# Autodesk Inventor assembly: MO-237
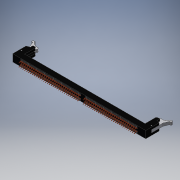
[picture p0: Inventor's stored thumbnail of the model, 180x180]
Saved by Autodesk Inventor 2016 (Build 200138000, 138)
## iProperties
Created: 2016-07-08
Part Number: MO-237
Document SubType Name: Assembly
Designer: Jonathan
Author: Jonathan
## Documents named in this file (4)
- C:\Users\Jonathan\Documents\Projects\mppcInterface\mppcInterface\cad\electronics\MO-237\MO-237.iam
- C:\Users\Jonathan\Documents\Projects\mppcInterface\mppcInterface\cad\electronics\MO-237\body.ipt
- C:\Users\Jonathan\Documents\Projects\mppcInterface\mppcInterface\cad\electronics\MO-237\pins.ipt
- C:\Users\Jonathan\Documents\Projects\mppcInterface\mppcInterface\cad\electronics\MO-237\pins2.ipt
## Components (241 placed, 3 different names)
1. body:1 — Mate:1, Mate:2, Mate:3, Mate:4, Mate:5, Mate:6, Mate:7, Mate:8, Mate:9, Mate:10, Mate:11, Mate:12, Mate:13, Mate:14, Mate:15, Mate:16
2. pins:1 — Mate:1, Mate:2
3. pins:2
4. pins:3
5. pins:4
6. pins:5
7. pins:6
8. pins:7
9. pins:8
10. pins:9
11. pins:10
12. pins:11
13. pins:12
14. pins:13
15. pins:14
16. pins:15
17. pins:16
18. pins:17
19. pins:18
20. pins:19
21. pins:20
22. pins:21
23. pins:22
24. pins:23
25. pins:24
26. pins:25
27. pins:26
28. pins:27
29. pins:28
30. pins:29
31. pins:30
32. pins:31
33. pins:32
34. pins:33 — Mate:3, Mate:4
35. pins:34
36. pins:35
37. pins:36
38. pins:37
39. pins:38
40. pins:39
41. pins:40
42. pins:41
43. pins:42
44. pins:43
45. pins:44
46. pins:45
47. pins:46
48. pins:47
49. pins:48
50. pins:49
51. pins:50
52. pins:51
53. pins:52
54. pins:53
55. pins:54
56. pins:55
57. pins:56
58. pins:57
59. pins:58
60. pins:59
61. pins:60
62. pins:61 — Mate:5, Mate:6
63. pins:62
64. pins:63
65. pins:64
66. pins:65
67. pins:66
68. pins:67
69. pins:68
70. pins:69
71. pins:70
72. pins:71
73. pins:72
74. pins:73
75. pins:74
76. pins:75
77. pins:76
78. pins:77
79. pins:78
80. pins:79
81. pins:80
82. pins:81
83. pins:82
84. pins:83
85. pins:84
86. pins:85
87. pins:86
88. pins:87
89. pins:88
90. pins:89
91. pins:90
92. pins:91
93. pins:92
94. pins:93 — Mate:7, Mate:8
95. pins:94
96. pins:95
97. pins:96
98. pins:97
99. pins:98
100. pins:99
101. pins:100
102. pins:101
103. pins:102
104. pins:103
105. pins:104
106. pins:105
107. pins:106
108. pins:107
109. pins:108
110. pins:109
111. pins:110
112. pins:111
113. pins:112
114. pins:113
115. pins:114
116. pins:115
117. pins:116
118. pins:117
119. pins:118
120. pins:119
121. pins:120
122. pins2:1 — Mate:9, Mate:10
123. pins2:5
124. pins2:6
125. pins2:7
126. pins2:8
127. pins2:9
128. pins2:10
129. pins2:11
130. pins2:12
131. pins2:13
132. pins2:14
133. pins2:15
134. pins2:16
135. pins2:17
136. pins2:18
137. pins2:19
138. pins2:20
139. pins2:21
140. pins2:22
141. pins2:23
142. pins2:24
143. pins2:25
144. pins2:26
145. pins2:27
146. pins2:28
147. pins2:29
148. pins2:30
149. pins2:31
150. pins2:2 — Mate:11, Mate:12
151. pins2:32
152. pins2:33
153. pins2:34
154. pins2:35
155. pins2:36
156. pins2:37
157. pins2:38
158. pins2:39
159. pins2:40
160. pins2:41
161. pins2:42
162. pins2:43
163. pins2:44
164. pins2:45
165. pins2:46
166. pins2:47
167. pins2:48
168. pins2:49
169. pins2:50
170. pins2:51
171. pins2:52
172. pins2:53
173. pins2:54
174. pins2:55
175. pins2:56
176. pins2:57
177. pins2:58
178. pins2:4 — Mate:13, Mate:14
179. pins2:59
180. pins2:60
181. pins2:61
182. pins2:62
183. pins2:63
184. pins2:64
185. pins2:65
186. pins2:66
187. pins2:67
188. pins2:68
189. pins2:69
190. pins2:70
191. pins2:71
192. pins2:72
193. pins2:73
194. pins2:74
195. pins2:75
196. pins2:76
197. pins2:77
198. pins2:78
199. pins2:79
200. pins2:80
201. pins2:81
202. pins2:82
203. pins2:83
204. pins2:84
205. pins2:85
206. pins2:86
207. pins2:87
208. pins2:88
209. pins2:89
210. pins2:3 — Mate:15, Mate:16
211. pins2:90
212. pins2:91
213. pins2:92
214. pins2:93
215. pins2:94
216. pins2:95
217. pins2:96
218. pins2:97
219. pins2:98
220. pins2:99
221. pins2:100
222. pins2:101
223. pins2:102
224. pins2:103
225. pins2:104
226. pins2:105
227. pins2:106
228. pins2:107
229. pins2:108
230. pins2:109
231. pins2:110
232. pins2:111
233. pins2:112
234. pins2:113
235. pins2:114
236. pins2:115
237. pins2:116
238. pins2:117
239. pins2:118
240. pins2:119
241. pins2:120
## Component patterns: (32 elements, first: pins:1), (28 elements, first: pins:33), (32 elements, first: pins:61), (28 elements, first: pins:93), (28 elements, first: pins2:1), (28 elements, first: pins2:2), (32 elements, first: pins2:4), (32 elements, first: pins2:3)
## Relationships (16: Mate 16)
- Mate:1: body:1 ↔ pins:1
- Mate:2: body:1 ↔ pins:1
- Mate:3: body:1 ↔ pins:33
- Mate:4: body:1 ↔ pins:33
- Mate:5: body:1 ↔ pins:61
- Mate:6: body:1 ↔ pins:61
- Mate:7: body:1 ↔ pins:93
- Mate:8: body:1 ↔ pins:93
- Mate:9: body:1 ↔ pins2:1
- Mate:10: body:1 ↔ pins2:1
- Mate:11: body:1 ↔ pins2:2
- Mate:12: body:1 ↔ pins2:2
- Mate:13: body:1 ↔ pins2:4
- Mate:14: body:1 ↔ pins2:4
- Mate:15: body:1 ↔ pins2:3
- Mate:16: body:1 ↔ pins2:3
